# Autodesk Inventor assembly: 203
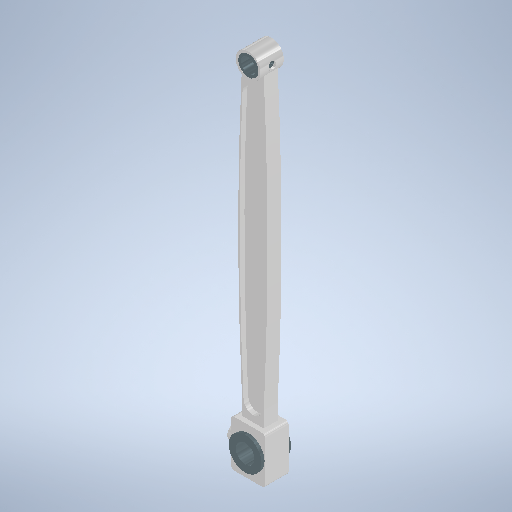
[picture p0: Inventor's stored thumbnail of the model, 512x512]
Saved by Autodesk Inventor 2025.1 (Build 291241000, 241)
## iProperties
Created: 2024-06-12
Part Number: 203
Document SubType Name: Assembly
Designer: ffogue
Author: ffogue
## Documents named in this file (4)
- C:\Users\ffogue\Downloads\Meine Projket\Paddle\203.iam
- C:\Users\ffogue\Downloads\Meine Projket\Paddle\2031.ipt
- C:\Users\ffogue\Downloads\Meine Projket\Paddle\2033.ipt
- C:\Users\ffogue\Downloads\Meine Projket\Paddle\2032.ipt
## Components (3 placed, 3 different names)
1. 2031:1 — Insert:1, Insert:2
2. 2032:1 — Insert:1
3. 2033:1 — Insert:2
## Relationships (2: Insert 2)
- Insert:1 (-15 mm): 2031:1 ↔ 2032:1
- Insert:2: 2031:1 ↔ 2033:1
